# Autodesk Inventor assembly: 後脚ギアトレイン5
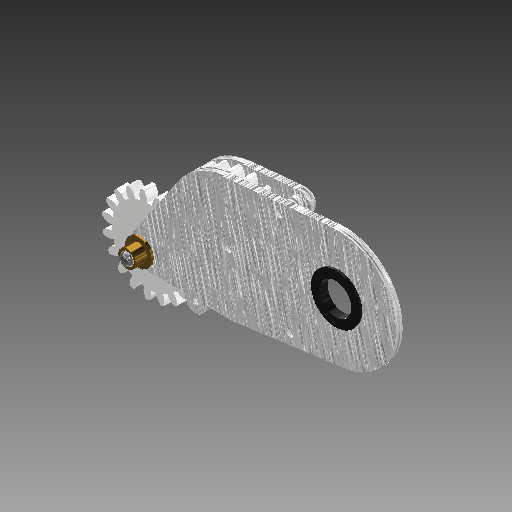
[picture p0: Inventor's stored thumbnail of the model, 512x512]
Saved by Autodesk Inventor 2020 (Build 240168000, 168)
## iProperties
Created: 2019-09-03
Part Number: 後脚ギアトレイン5
Document SubType Name: Assembly
Designer: 雪村
Mass: 102.652 g
Surface Area: 323.697 cm^2
Volume: 41.3618 cm^3
Density: 2.4818 g/cm^3
Author: 雪村
## Documents named in this file (11)
- C:\Users\white\Documents\SRDC\SRDC\Inventor_2017\2018年機体\2020年4年機体\後脚ギアトレイン5.iam
- C:\Users\white\Documents\SRDC\SRDC\Inventor_2017\2018年機体\2020年4年機体\後脚ギアトレイン5.1.ipt
- C:\Users\white\Documents\SRDC\SRDC\Inventor_2017\2018年機体\2020年4年機体\後脚ギアトレイン5.2.ipt
- C:\Users\white\Documents\SRDC\SRDC\Inventor_2017\2018年機体\パーツ\スペーサーm3,7.ipt
- C:\Users\white\Documents\SRDC\SRDC\Inventor_2017\2018年機体\2020年4年機体\歯車m2.z19.ipt
- C:\Users\white\Documents\SRDC\SRDC\Inventor_2017\2018年機体\パーツ\ベアリングフランジ付き0610.3t.ipt
- C:\Users\white\Documents\SRDC\SRDC\Inventor_2017\2018年機体\2020年4年機体\歯車m2.z25.ipt
- C:\Users\white\Documents\SRDC\SRDC\Inventor_2017\2018年機体\パーツ\オイレスフランジ付き06080512,1t ドライメット.ipt
- C:\Users\white\Documents\SRDC\SRDC\Inventor_2017\2018年機体\パーツ\スペーサーm3,6.ipt
- C:\Users\white\Documents\SRDC\SRDC\Inventor_2017\2018年機体\パーツ\ネジ鍋m3,12.ipt
- C:\Users\white\Documents\SRDC\SRDC\Inventor_2017\2018年機体\パーツ\オイレスフランジ付き14162202.5.ipt
## Components (20 placed, 10 different names)
1. 後脚ギアトレイン5.1:1 — 挿入:1, 挿入:2, 挿入:3, 挿入:6, 挿入:9, 挿入:12, 挿入:16, 挿入:20
2. 後脚ギアトレイン5.2:1 — 挿入:13, メイト:1, 挿入:18
3. スペーサーm3,7:1 — 挿入:1
4. スペーサーm3,7:2 — 挿入:6, メイト:1
5. スペーサーm3,7:4 — 挿入:2, 挿入:13
6. スペーサーm3,7:5
7. スペーサーm3,7:6 — 挿入:3
8. 歯車m2.z19:1
9. ベアリングフランジ付き0610.3t:1 — 挿入:9
10. ベアリングフランジ付き0610.3t:2
11. 歯車m2.z25:1 — 挿入:10, 挿入:11
12. ベアリングフランジ付き0610.3t:3 — 挿入:10, 挿入:12
13. ベアリングフランジ付き0610.3t:4 — 挿入:11
14. オイレスフランジ付き06080512,1t ドライメット:1 — 挿入:18, 挿入:19
15. オイレスフランジ付き06080512,1t ドライメット:2 — 挿入:17
16. スペーサーm3,6:1 — 挿入:19
17. スペーサーm3,6:2 — 挿入:16, 挿入:17
18. ネジ鍋m3,12:1
19. ネジ鍋m3,12:2
20. オイレスフランジ付き14162202.5:1 — 挿入:20
## Relationships (19: Insert 18, Mate 1)
- 挿入:1 [Insert]: 後脚ギアトレイン5.1:1 ↔ スペーサーm3,7:1
- 挿入:2 [Insert]: 後脚ギアトレイン5.1:1 ↔ スペーサーm3,7:4
- 挿入:3 [Insert]: 後脚ギアトレイン5.1:1 ↔ スペーサーm3,7:6
- 挿入:6 [Insert]: 後脚ギアトレイン5.1:1 ↔ スペーサーm3,7:2
- [Insert]: 歯車m2.z19:1 ↔ ベアリングフランジ付き0610.3t:1
- [Insert]: 歯車m2.z19:1 ↔ ベアリングフランジ付き0610.3t:2
- 挿入:9 [Insert]: 後脚ギアトレイン5.1:1 ↔ ベアリングフランジ付き0610.3t:1
- 挿入:10 [Insert]: 歯車m2.z25:1 ↔ ベアリングフランジ付き0610.3t:3
- 挿入:11 [Insert]: 歯車m2.z25:1 ↔ ベアリングフランジ付き0610.3t:4
- 挿入:12 [Insert]: 後脚ギアトレイン5.1:1 ↔ ベアリングフランジ付き0610.3t:3
- 挿入:13 [Insert]: 後脚ギアトレイン5.2:1 ↔ スペーサーm3,7:4
- メイト:1 [Mate]: 後脚ギアトレイン5.2:1 ↔ スペーサーm3,7:2
- [Insert]: オイレスフランジ付き06080512,1t ドライメット:1 ↔ ネジ鍋m3,12:1
- [Insert]: スペーサーm3,6:2 ↔ ネジ鍋m3,12:2
- 挿入:16 [Insert]: 後脚ギアトレイン5.1:1 ↔ スペーサーm3,6:2
- 挿入:17 [Insert]: オイレスフランジ付き06080512,1t ドライメット:2 ↔ スペーサーm3,6:2
- 挿入:18 [Insert]: 後脚ギアトレイン5.2:1 ↔ オイレスフランジ付き06080512,1t ドライメット:1
- 挿入:19 [Insert]: オイレスフランジ付き06080512,1t ドライメット:1 ↔ スペーサーm3,6:1
- 挿入:20 [Insert]: 後脚ギアトレイン5.1:1 ↔ オイレスフランジ付き14162202.5:1
## Named parameters: d6_d1 = 0 mm, d7_d0 = 0 mm
